# Autodesk Inventor assembly: Ensamble
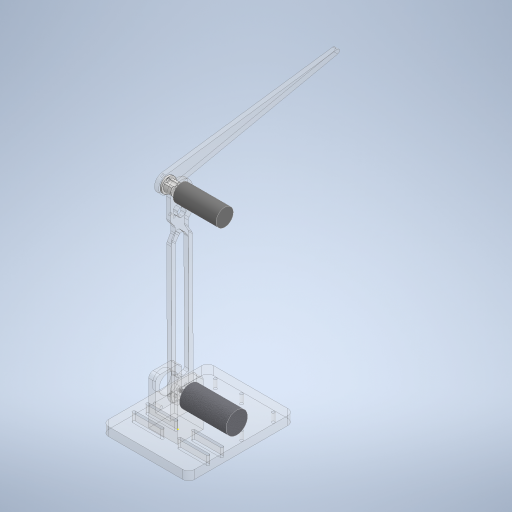
[picture p0: Inventor's stored thumbnail of the model, 512x512]
Saved by Autodesk Inventor 2024 (Build 280153000, 153)
## iProperties
Created: 2024-08-26
Part Number: Ensamble
Document SubType Name: Assembly
Designer: David Ricaurte
Author: David Ricaurte
## Documents named in this file (8)
- C:\Users\David Ricaurte\Documents\servos\2ver\Ensamble.iam
- C:\Users\David Ricaurte\Documents\servos\2ver\base.ipt
- C:\Users\David Ricaurte\Documents\servos\motor.ipt
- C:\Users\David Ricaurte\Documents\servos\motor2.ipt
- C:\Users\David Ricaurte\Documents\servos\2ver\acople.ipt
- C:\Users\David Ricaurte\Documents\servos\2ver\puntero.ipt
- C:\Users\David Ricaurte\Documents\servos\2ver\Part51.ipt
- C:\Users\David Ricaurte\Documents\servos\2ver\bas.ipt
## Components (7 placed, 7 different names)
1. base:1 — Insert:1, Mate:1, Flush:1
2. motor:1 — Insert:1, Rotational:1
3. motor2:1 — Insert:4, Rotational:2
4. acople:1 — Insert:2, Insert:3, Rotational:2
5. puntero:1 — Insert:2, Insert:3
6. Part51:1 — Insert:4, Rotational:1
7. bas:1 — Mate:1, Flush:1
## Relationships (8: Insert 4, RevoluteJoint 2, Mate 1, Flush 1)
- Insert:1: base:1 ↔ motor:1
- Insert:2: acople:1 ↔ puntero:1
- Insert:3: acople:1 ↔ puntero:1
- Insert:4: motor2:1 ↔ Part51:1
- Rotational:1 [RevoluteJoint] (-2 mm): motor:1 ↔ Part51:1
- Rotational:2 [RevoluteJoint] (-2 mm): motor2:1 ↔ acople:1
- Mate:1: base:1 ↔ bas:1
- Flush:1 (-22 mm): base:1 ↔ bas:1
